# Autodesk Inventor assembly: Assembly1
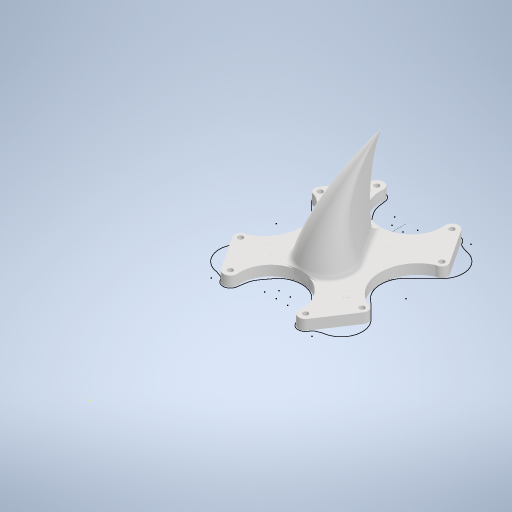
[picture p0: Inventor's stored thumbnail of the model, 512x512]
Saved by Autodesk Inventor 2023 (Build 270158000, 158)
## iProperties
Created: 2023-01-26
Part Number: Assembly1
Document SubType Name: Assembly
Designer: Steven
Author: Steven
## Documents named in this file (3)
- Y:\FPV drone stuff\0 Street League\Frames\experimental-quad-frames\Nightstick MAX\3D prints\shark fin experiments\Assembly1.iam
- Y:\FPV drone stuff\0 Street League\Frames\experimental-quad-frames\Nightstick MAX\3D prints\shark fin experiments\Part1.ipt
- Y:\FPV drone stuff\0 Street League\Frames\experimental-quad-frames\Nightstick MAX\3D prints\shark fin experiments\Shark fin.ipt
## Components (2 placed, 2 different names)
1. Part1:1 — Flush:1, Flush:2, Flush:3, Flush:4, Flush:5
2. Shark fin:1 — Flush:4, Flush:5
## Relationships (5: Flush 5)
- Flush:1: Part1:1
- Flush:2: Part1:1
- Flush:3: Part1:1
- Flush:4: Part1:1 ↔ Shark fin:1
- Flush:5: Part1:1 ↔ Shark fin:1
